# Autodesk Inventor assembly: Ensamblaje Proyecto IOT
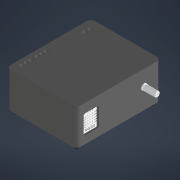
[picture p0: Inventor's stored thumbnail of the model, 180x180]
Saved by Autodesk Inventor 2021 (Build 250183000, 183)
## iProperties
Created: 2021-03-29
Part Number: Ensamblaje Proyecto IOT
Document SubType Name: Assembly
Designer: grego
Author: grego
## Documents named in this file (5)
- C:\Users\grego\Desktop\Ensamblaje Proyecto IOT.iam
- C:\Users\grego\Desktop\Case Proyecto IOT.ipt
- D:\ESPE\7mo Semestre\Diseño Electrónico\Tercer Parcial\IOT ESP8266\Circuito y PCB\Proyecto IOT.ipt
- C:\Users\grego\Desktop\Tapa Case.ipt
- C:\Users\grego\Desktop\Soportes.ipt
## Components (7 placed, 4 different names)
1. Case Proyecto IOT:1 — Coincidencia:1, Coincidencia:2, Coincidencia:3, Coincidencia:4, Nivelación:1, Nivelación:2, Coincidencia:5, Coincidencia:6, Coincidencia:7, Coincidencia:8, Coincidencia:9, Coincidencia:10, Coincidencia:11, Coincidencia:12
2. Proyecto IOT:1 — Coincidencia:1, Coincidencia:2, Coincidencia:3
3. Tapa Case:1 — Coincidencia:4, Nivelación:1, Nivelación:2
4. Soportes:1 — Coincidencia:5, Coincidencia:6
5. Soportes:2 — Coincidencia:7, Coincidencia:8
6. Soportes:3 — Coincidencia:9, Coincidencia:10
7. Soportes:4 — Coincidencia:11, Coincidencia:12
## Relationships (14: Mate 12, Flush 2)
- Coincidencia:1 [Mate]: Case Proyecto IOT:1 ↔ Proyecto IOT:1
- Coincidencia:2 [Mate]: Case Proyecto IOT:1 ↔ Proyecto IOT:1
- Coincidencia:3 [Mate]: Case Proyecto IOT:1 ↔ Proyecto IOT:1
- Coincidencia:4 [Mate]: Case Proyecto IOT:1 ↔ Tapa Case:1
- Nivelación:1 [Flush]: Case Proyecto IOT:1 ↔ Tapa Case:1
- Nivelación:2 [Flush]: Case Proyecto IOT:1 ↔ Tapa Case:1
- Coincidencia:5 [Mate]: Case Proyecto IOT:1 ↔ Soportes:1
- Coincidencia:6 [Mate]: Case Proyecto IOT:1 ↔ Soportes:1
- Coincidencia:7 [Mate]: Case Proyecto IOT:1 ↔ Soportes:2
- Coincidencia:8 [Mate]: Case Proyecto IOT:1 ↔ Soportes:2
- Coincidencia:9 [Mate]: Case Proyecto IOT:1 ↔ Soportes:3
- Coincidencia:10 [Mate]: Case Proyecto IOT:1 ↔ Soportes:3
- Coincidencia:11 [Mate]: Case Proyecto IOT:1 ↔ Soportes:4
- Coincidencia:12 [Mate]: Case Proyecto IOT:1 ↔ Soportes:4
